# Autodesk Inventor assembly: FullRadiusPoleAJB
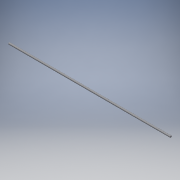
[picture p0: Inventor's stored thumbnail of the model, 180x180]
Saved by Autodesk Inventor 2018 (Build 220112000, 112)
## iProperties
Created: 2018-02-16
Part Number: FullRadiusPoleAJB
Document SubType Name: Assembly
Designer: Alec temporary
Author: Alec temporary
## Documents named in this file (3)
- M:\TPS\9th Grade\CADD 2017-2018\Current\Ferris Wheel Group Project\Group Project Week 3\FullRadiusPoleAJB.iam
- M:\TPS\9th Grade\CADD 2017-2018\Current\Ferris Wheel Group Project\Group Project Week 2b\Alec\1_6RadiusPole_WithBolt_AJB.iam
- M:\TPS\9th Grade\CADD 2017-2018\Current\Ferris Wheel Group Project\Group Project Week 2b\Alec\OuterRadiusPoleAJB.ipt
## Components (7 placed, 2 different names)
1. 1_6RadiusPole_WithBolt_AJB:1 [sub-assembly] — Mate:1, Mate:2, Mate:3, Mate:8
2. 1_6RadiusPole_WithBolt_AJB:2 [sub-assembly] — Mate:4, Mate:10, Mate:12
3. 1_6RadiusPole_WithBolt_AJB:3 [sub-assembly] — Mate:6, Mate:11, Mate:13, Mate:14
4. 1_6RadiusPole_WithBolt_AJB:4 [sub-assembly] — Mate:7, Mate:8, Mate:9
5. 1_6RadiusPole_WithBolt_AJB:5 [sub-assembly] — Mate:5, Mate:7, Mate:11, Mate:12
6. 1_6RadiusPole_WithBolt_AJB:6 [sub-assembly] — Mate:3, Mate:4, Mate:5, Mate:6, Mate:9, Mate:10
7. OuterRadiusPoleAJB:1 — Mate:13, Mate:14
## Relationships (14: Mate 14)
- Mate:1: 1_6RadiusPole_WithBolt_AJB:1
- Mate:2: 1_6RadiusPole_WithBolt_AJB:1
- Mate:3: 1_6RadiusPole_WithBolt_AJB:1 ↔ 1_6RadiusPole_WithBolt_AJB:6
- Mate:4: 1_6RadiusPole_WithBolt_AJB:2 ↔ 1_6RadiusPole_WithBolt_AJB:6
- Mate:5: 1_6RadiusPole_WithBolt_AJB:5 ↔ 1_6RadiusPole_WithBolt_AJB:6
- Mate:6: 1_6RadiusPole_WithBolt_AJB:3 ↔ 1_6RadiusPole_WithBolt_AJB:6
- Mate:7: 1_6RadiusPole_WithBolt_AJB:4 ↔ 1_6RadiusPole_WithBolt_AJB:5
- Mate:8: 1_6RadiusPole_WithBolt_AJB:1 ↔ 1_6RadiusPole_WithBolt_AJB:4
- Mate:9: 1_6RadiusPole_WithBolt_AJB:4 ↔ 1_6RadiusPole_WithBolt_AJB:6
- Mate:10: 1_6RadiusPole_WithBolt_AJB:2 ↔ 1_6RadiusPole_WithBolt_AJB:6
- Mate:11: 1_6RadiusPole_WithBolt_AJB:3 ↔ 1_6RadiusPole_WithBolt_AJB:5
- Mate:12: 1_6RadiusPole_WithBolt_AJB:2 ↔ 1_6RadiusPole_WithBolt_AJB:5
- Mate:13: 1_6RadiusPole_WithBolt_AJB:3 ↔ OuterRadiusPoleAJB:1
- Mate:14: 1_6RadiusPole_WithBolt_AJB:3 ↔ OuterRadiusPoleAJB:1
